# Autodesk Inventor assembly: Assembly
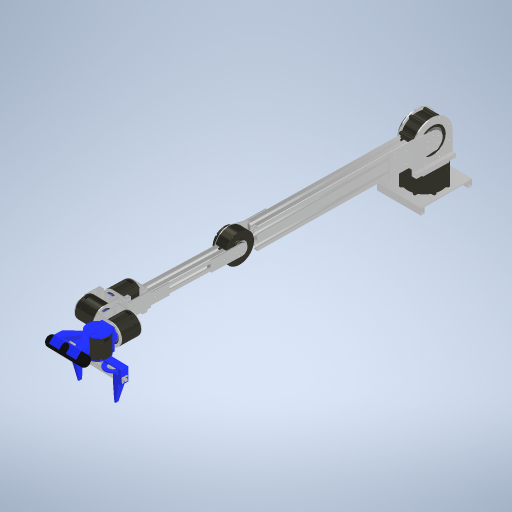
[picture p0: Inventor's stored thumbnail of the model, 512x512]
Saved by Autodesk Inventor 2024 (Build 280153000, 153)
## iProperties
Created: 2024-12-13
Part Number: Assembly
Document SubType Name: Assembly
Designer: hirek
Mass: 4906.56 g
Surface Area: 10894.8 cm^2
Volume: 1127.79 cm^3
Density: 4.35059 g/cm^3
Author: hirek
## Documents named in this file (13)
- E:\Documents\Inventor\CanAloha\Assembly.iam
- E:\Documents\Inventor\CanAloha\Link1.iam
- E:\Documents\Inventor\CanAloha\Link2.iam
- E:\Documents\Inventor\CanAloha\Link3.iam
- E:\Documents\Inventor\CanAloha\Link4.iam
- E:\Documents\Inventor\CanAloha\Link5.iam
- E:\Documents\Inventor\CanAloha\EndEff.iam
- E:\Documents\Inventor\CanAloha\Assembly\AIP\FEA\ex44crew0.fins
- E:\Documents\Inventor\CanAloha\Assembly\AIP\FEA\ex44crew0.fsat
- E:\Documents\Inventor\CanAloha\Assembly\AIP\FEA\ex44crew0.ftes
- E:\Documents\Inventor\CanAloha\Assembly\AIP\FEA\ex44crew0.fwiz
- E:\Documents\Inventor\CanAloha\Assembly\AIP\FEA\ex44crf8g.fmsh
- E:\Documents\Inventor\CanAloha\Assembly\AIP\FEA\ex44crf8h.fres
## Components (7 placed, 6 different names)
1. Link1:1 [sub-assembly] — 回転:1
2. Link2:1 [sub-assembly] — 回転:1, 回転:2
3. Link3:1 [sub-assembly] — 回転:2, 挿入:1
4. Link4:1 [sub-assembly] — 挿入:1, 挿入:2
5. Link5:1 [sub-assembly] — 挿入:2, 挿入:3
6. Link5:2 [sub-assembly] — 挿入:3, 挿入:4
7. EndEff:1 [sub-assembly] — 挿入:4
## Relationships (6: Insert 4, RevoluteJoint 2)
- 回転:1 [RevoluteJoint]: Link1:1 ↔ Link2:1
- 回転:2 [RevoluteJoint]: Link2:1 ↔ Link3:1
- 挿入:1 [Insert]: Link3:1 ↔ Link4:1
- 挿入:2 [Insert]: Link4:1 ↔ Link5:1
- 挿入:3 [Insert]: Link5:1 ↔ Link5:2
- 挿入:4 [Insert]: Link5:2 ↔ EndEff:1
